# Autodesk Inventor assembly: bubble-wall
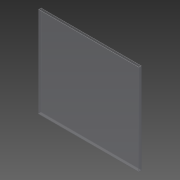
[picture p0: Inventor's stored thumbnail of the model, 180x180]
Saved by Autodesk Inventor 2013 (Build 170138000, 138)
## iProperties
Created: 2013-04-25
Part Number: bubble-wall
Document SubType Name: Assembly
Designer: Chris
Author: Chris
## Documents named in this file (4)
- C:\Users\Chris\Documents\Inventor\Redbull-2013\bubble-wall\bubble-wall.iam
- C:\Users\Chris\Documents\Inventor\Redbull-2013\bubble-wall\bottom-panel.ipt
- C:\Users\Chris\Documents\Inventor\Redbull-2013\bubble-wall\front-panel.ipt
- C:\Users\Chris\Documents\Inventor\Redbull-2013\bubble-wall\side-panel.ipt
## Components (5 placed, 3 different names)
1. bottom-panel:1 — Flush:1, Mate:1, Flush:2, Mate:2, Flush:3, Flush:4, Mate:3, Flush:5, Flush:6, Mate:4, Flush:7, Flush:8
2. front-panel:1 — Flush:1, Mate:1, Flush:2
3. front-panel:2 — Mate:2, Flush:3, Flush:4
4. side-panel:1 — Mate:3, Flush:5, Flush:6
5. side-panel:2 — Mate:4, Flush:7, Flush:8
## Relationships (12: Flush 8, Mate 4)
- Flush:1: bottom-panel:1 ↔ front-panel:1
- Mate:1: bottom-panel:1 ↔ front-panel:1
- Flush:2 (6.35 mm): bottom-panel:1 ↔ front-panel:1
- Mate:2: bottom-panel:1 ↔ front-panel:2
- Flush:3: bottom-panel:1 ↔ front-panel:2
- Flush:4 (6.35 mm): bottom-panel:1 ↔ front-panel:2
- Mate:3: bottom-panel:1 ↔ side-panel:1
- Flush:5: bottom-panel:1 ↔ side-panel:1
- Flush:6: bottom-panel:1 ↔ side-panel:1
- Mate:4: bottom-panel:1 ↔ side-panel:2
- Flush:7: bottom-panel:1 ↔ side-panel:2
- Flush:8: bottom-panel:1 ↔ side-panel:2
